# Autodesk Inventor assembly: CAR_034_KickerAssembly
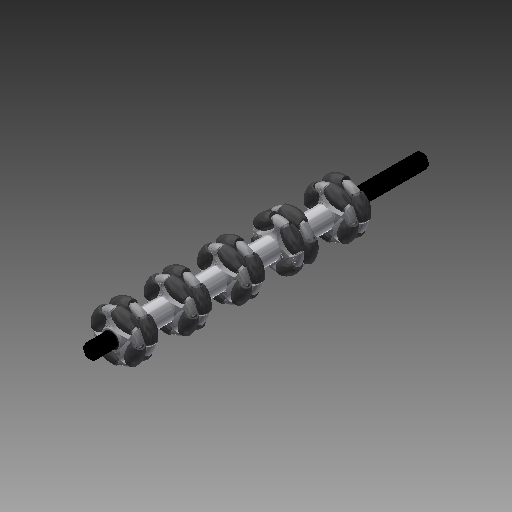
[picture p0: Inventor's stored thumbnail of the model, 512x512]
Saved by Autodesk Inventor 2018.3 (Build 223284000, 284)
## iProperties
Created: 2020-02-07
Part Number: CAR_034_KickerAssembly
Document SubType Name: Assembly
Designer: jd2
Author: jd2
## Documents named in this file (4)
- C:\Users\22barlalex\Documents\GrabCAD\Infinite Recharge 2020\Build season\CAR_034_SweeperBarAssembly.iam
- C:\Users\22barlalex\Documents\GrabCAD\Infinite Recharge 2020\Build season\CAR_035_Sweeper12inHexShaft.ipt
- C:\Users\22barlalex\Documents\GrabCAD\Infinite Recharge 2020\Build season\CAR_037_2inOmniWheel.iam
- C:\Users\22barlalex\Documents\GrabCAD\Infinite Recharge 2020\Build season\CAR_39_1inchSpacers.ipt
## Components (10 placed, 3 different names)
1. CAR_035_Sweeper12inHexShaft:1 — Mate:1, Mate:2, Mate:3, Mate:4, Mate:5, Mate:6, Mate:7, Mate:8, Mate:14, Mate:15
2. CAR_037_2inOmniWheel:1 [sub-assembly] — Mate:1, Mate:5, Mate:11
3. CAR_037_2inOmniWheel:2 [sub-assembly] — Mate:2, Mate:6, Mate:11, Mate:12, Insert:1
4. CAR_037_2inOmniWheel:3 [sub-assembly] — Mate:3, Mate:7, Mate:12, Mate:13, Insert:2
5. CAR_037_2inOmniWheel:4 [sub-assembly] — Mate:4, Mate:8, Mate:13, Insert:3, Mate:16
6. CAR_39_1inchSpacers:1 — Insert:1
7. CAR_39_1inchSpacers:2 — Insert:2
8. CAR_39_1inchSpacers:3 — Insert:3
9. CAR_037_2inOmniWheel:6 [sub-assembly] — Mate:14, Mate:15, Mate:16, Insert:4
10. CAR_39_1inchSpacers:4 — Insert:4
## Relationships (18: Mate 14, Insert 4)
- Mate:1: CAR_035_Sweeper12inHexShaft:1 ↔ CAR_037_2inOmniWheel:1
- Mate:2: CAR_035_Sweeper12inHexShaft:1 ↔ CAR_037_2inOmniWheel:2
- Mate:3: CAR_035_Sweeper12inHexShaft:1 ↔ CAR_037_2inOmniWheel:3
- Mate:4: CAR_035_Sweeper12inHexShaft:1 ↔ CAR_037_2inOmniWheel:4
- Mate:5: CAR_035_Sweeper12inHexShaft:1 ↔ CAR_037_2inOmniWheel:1
- Mate:6: CAR_035_Sweeper12inHexShaft:1 ↔ CAR_037_2inOmniWheel:2
- Mate:7: CAR_035_Sweeper12inHexShaft:1 ↔ CAR_037_2inOmniWheel:3
- Mate:8: CAR_035_Sweeper12inHexShaft:1 ↔ CAR_037_2inOmniWheel:4
- Mate:11 (25.4 mm): CAR_037_2inOmniWheel:1 ↔ CAR_037_2inOmniWheel:2
- Mate:12 (25.4 mm): CAR_037_2inOmniWheel:2 ↔ CAR_037_2inOmniWheel:3
- Mate:13 (25.4 mm): CAR_037_2inOmniWheel:3 ↔ CAR_037_2inOmniWheel:4
- Insert:1: CAR_037_2inOmniWheel:2 ↔ CAR_39_1inchSpacers:1
- Insert:2: CAR_037_2inOmniWheel:3 ↔ CAR_39_1inchSpacers:2
- Insert:3: CAR_037_2inOmniWheel:4 ↔ CAR_39_1inchSpacers:3
- Mate:14: CAR_035_Sweeper12inHexShaft:1 ↔ CAR_037_2inOmniWheel:6
- Mate:15: CAR_035_Sweeper12inHexShaft:1 ↔ CAR_037_2inOmniWheel:6
- Mate:16 (25.4 mm): CAR_037_2inOmniWheel:4 ↔ CAR_037_2inOmniWheel:6
- Insert:4: CAR_037_2inOmniWheel:6 ↔ CAR_39_1inchSpacers:4
